# Autodesk Inventor assembly: Mecanum_Assembly
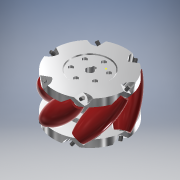
[picture p0: Inventor's stored thumbnail of the model, 180x180]
Saved by Autodesk Inventor 2018 (Build 220112000, 112)
## iProperties
Created: 2017-09-05
Part Number: Mecanum_Assembly
Document SubType Name: Assembly
Designer: P136265
Author: P136265
## Documents named in this file (8)
- C:\Users\P136265\Documents\mecanum-cad\Mecanum_Assembly.iam
- C:\Users\P136265\Documents\mecanum-cad\roller 8-19-6 bearing.ipt
- C:\Users\P136265\Documents\Inventor\Content Center Files\R2018\en-US\DIN 625 SKF(4)\DIN 625 SKF - SKF 619_8-2Z.ipt
- C:\Users\P136265\Documents\mecanum-cad\MecanumShaft.ipt
- C:\Users\P136265\Documents\mecanum-cad\PE_Sleeve.ipt
- C:\Users\P136265\Documents\mecanum-cad\CheekPlate.ipt
- C:\Users\P136265\Documents\mecanum-cad\MecanumHub.ipt
- C:\Users\P136265\Documents\mecanum-cad\Washer.ipt
## Components (45 placed, 7 different names)
1. CheekPlate:1 — Angle:10, Angle:11, Mate:19, Angle:12, Mate:20, Mate:21, Angle:13, Angle:14
2. MecanumHub:1 — Angle:12, Mate:20, Mate:21, Mate:22
3. CheekPlate:2 — Angle:13, Angle:14, Angle:15, Mate:22, Mate:23
4. roller 8-19-6 bearing:1 — Mate:1, Angle:1, Mate:2, Angle:11
5. roller 8-19-6 bearing:2
6. roller 8-19-6 bearing:3 — Insert:1, Insert:2, Angle:8, Angle:9
7. roller 8-19-6 bearing:4 — Angle:2, Mate:3, Mate:4
8. roller 8-19-6 bearing:5
9. roller 8-19-6 bearing:6
10. DIN 625 SKF- with two Z shields SKF 619/8-2Z:1 — Insert:1, Mate:17
11. DIN 625 SKF- with two Z shields SKF 619/8-2Z:3
12. DIN 625 SKF- with two Z shields SKF 619/8-2Z:4
13. DIN 625 SKF- with two Z shields SKF 619/8-2Z:5
14. DIN 625 SKF- with two Z shields SKF 619/8-2Z:6
15. DIN 625 SKF- with two Z shields SKF 619/8-2Z:7
16. DIN 625 SKF- with two Z shields SKF 619/8-2Z:2 — Insert:2, Mate:15
17. DIN 625 SKF- with two Z shields SKF 619/8-2Z:8 — Flush:1
18. DIN 625 SKF- with two Z shields SKF 619/8-2Z:9
19. DIN 625 SKF- with two Z shields SKF 619/8-2Z:10
20. DIN 625 SKF- with two Z shields SKF 619/8-2Z:11
21. DIN 625 SKF- with two Z shields SKF 619/8-2Z:12
22. MecanumShaft:1 — Angle:2, Mate:3, Flush:1, Angle:3, Angle:15, Mate:23
23. MecanumShaft:2
24. MecanumShaft:3
25. MecanumShaft:4
26. MecanumShaft:5
27. MecanumShaft:6 — Mate:16, Mate:18, Angle:10
28. PE_Sleeve:1 — Angle:3, Mate:4
29. PE_Sleeve:2
30. PE_Sleeve:3
31. PE_Sleeve:4
32. PE_Sleeve:5
33. PE_Sleeve:6
34. Washer:2 — Angle:9, Mate:17, Mate:18
35. Washer:1 — Angle:8, Mate:15, Mate:16
36. Washer:3
37. Washer:4
38. Washer:5
39. Washer:6
40. Washer:7
41. Washer:8
42. Washer:9 — Mate:19
43. Washer:10
44. Washer:11
45. Washer:12
## Component patterns: (6 elements, first: roller 8-19-6 bearing:1), (6 elements, first: DIN 625 SKF- with two Z shields SKF 619/8-2Z:1), (6 elements, first: DIN 625 SKF- with two Z shields SKF 619/8-2Z:2), (6 elements, first: MecanumShaft:1), (6 elements, first: PE_Sleeve:1), (6 elements, first: Washer:2 + Washer:1)
## Relationships (27: Mate 13, Angle 11, Insert 2, Flush 1)
- Mate:1 (75 mm): roller 8-19-6 bearing:1
- Angle:1 (45 deg): roller 8-19-6 bearing:1
- Mate:2: roller 8-19-6 bearing:1
- Insert:1: roller 8-19-6 bearing:3 ↔ DIN 625 SKF- with two Z shields SKF 619/8-2Z:1
- Insert:2: roller 8-19-6 bearing:3 ↔ DIN 625 SKF- with two Z shields SKF 619/8-2Z:2
- Angle:2 (0 deg): roller 8-19-6 bearing:4 ↔ MecanumShaft:1
- Mate:3: roller 8-19-6 bearing:4 ↔ MecanumShaft:1
- Flush:1 (-20 mm): DIN 625 SKF- with two Z shields SKF 619/8-2Z:8 ↔ MecanumShaft:1
- Angle:3 (0 deg): MecanumShaft:1 ↔ PE_Sleeve:1
- Mate:4: roller 8-19-6 bearing:4 ↔ PE_Sleeve:1
- Angle:8 (0 deg): roller 8-19-6 bearing:3 ↔ Washer:1
- Mate:15: DIN 625 SKF- with two Z shields SKF 619/8-2Z:2 ↔ Washer:1
- Mate:16: MecanumShaft:6 ↔ Washer:1
- Angle:9 (0 deg): roller 8-19-6 bearing:3 ↔ Washer:2
- Mate:17: DIN 625 SKF- with two Z shields SKF 619/8-2Z:1 ↔ Washer:2
- Mate:18: MecanumShaft:6 ↔ Washer:2
- Angle:10 (0 deg): CheekPlate:1 ↔ MecanumShaft:6
- Angle:11 (0 deg): CheekPlate:1 ↔ roller 8-19-6 bearing:1
- Mate:19: CheekPlate:1 ↔ Washer:9
- Angle:12 (0 deg): CheekPlate:1 ↔ MecanumHub:1
- Mate:20: CheekPlate:1 ↔ MecanumHub:1
- Mate:21: CheekPlate:1 ↔ MecanumHub:1
- Angle:13 (0 deg): CheekPlate:1 ↔ CheekPlate:2
- Angle:14 (0 deg): CheekPlate:1 ↔ CheekPlate:2
- Angle:15 (0 deg): CheekPlate:2 ↔ MecanumShaft:1
- Mate:22: MecanumHub:1 ↔ CheekPlate:2
- Mate:23: CheekPlate:2 ↔ MecanumShaft:1
